# Autodesk Inventor assembly: Pedale
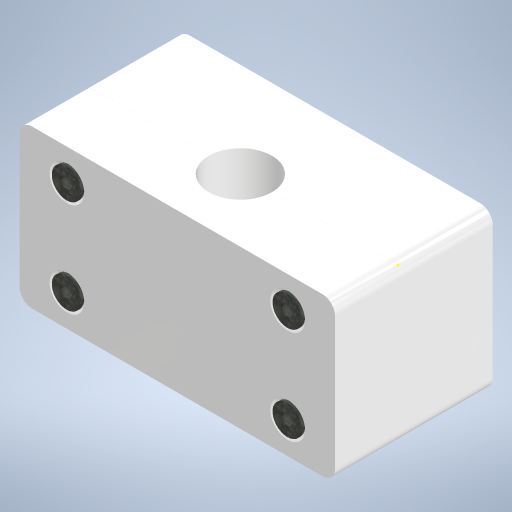
[picture p0: Inventor's stored thumbnail of the model, 512x512]
Saved by Autodesk Inventor 2024.4 (Build 284460000, 460)
## iProperties
Created: 2026-01-10
Part Number: Pedale
Description: Pedale
Document SubType Name: Assembly
Designer: Philf
Mass: 329.768 g
Surface Area: 413.976 cm^2
Volume: 234.145 cm^3
Density: 1.4084 g/cm^3
Masse[kg]: 0,330 kg
Author: Philf
## Documents named in this file (4)
- C:\Users\Philf\Documents\Vault\Daten\I60-Konstruktion\I60-Gruppe-7\Tritt\Pedale.iam
- C:\Users\Philf\Documents\Vault\Daten\I60-Konstruktion\I60-Gruppe-7\Tritt\TrittUT.ipt
- C:\Users\Philf\Documents\Vault\Daten\I60-Konstruktion\I60-Gruppe-7\Tritt\TrittOT.ipt
- C:\Users\Philf\Documents\Vault\Normteile\de-DE\ISO 10642(2)\ISO 10642  - M5  x  50.ipt
## Components (6 placed, 3 different names)
1. TrittUT:1 — Passend:1, Fluchtend:1, Fluchtend:2
2. TrittOT:1 — Passend:1, Fluchtend:1, Fluchtend:2, Passend:2, Passend:3, Passend:4, Passend:5
3. DIN EN ISO 10642 M5  x  50:1 — Passend:2
4. DIN EN ISO 10642 M5  x  50:2 — Passend:3
5. DIN EN ISO 10642 M5  x  50:3 — Passend:4
6. DIN EN ISO 10642 M5  x  50:4 — Passend:5
## Relationships (7: Mate 5, Flush 2)
- Passend:1 [Mate]: TrittUT:1 ↔ TrittOT:1
- Fluchtend:1 [Flush]: TrittUT:1 ↔ TrittOT:1
- Fluchtend:2 [Flush]: TrittUT:1 ↔ TrittOT:1
- Passend:2 [Mate]: TrittOT:1 ↔ DIN EN ISO 10642 M5  x  50:1
- Passend:3 [Mate]: TrittOT:1 ↔ DIN EN ISO 10642 M5  x  50:2
- Passend:4 [Mate]: TrittOT:1 ↔ DIN EN ISO 10642 M5  x  50:3
- Passend:5 [Mate]: TrittOT:1 ↔ DIN EN ISO 10642 M5  x  50:4
